# Autodesk Inventor assembly: Linear slides
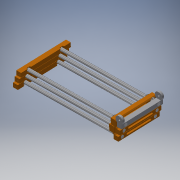
[picture p0: Inventor's stored thumbnail of the model, 180x180]
Saved by Autodesk Inventor 2019 (Build 230136000, 136)
## iProperties
Created: 2019-03-07
Part Number: Linear slides
Document SubType Name: Assembly
Designer: Delta
Mass: 697.362 g
Surface Area: 1389.66 cm^2
Volume: 258.282 cm^3
Density: 2.7 g/cm^3
Author: Delta
## Documents named in this file (6)
- C:\Robotics\2019-20_CAD\Linear Slides\Linear slides.iam
- C:\Robotics\2019-20_CAD\Linear Slides\Block_3-8.ipt
- C:\Robotics\2019-20_CAD\Linear Slides\rod_3-8_12 inch.ipt
- C:\Robotics\COTSParts\Bearings - McMaster\60595K120_FIXED ALIGNMENT  LINEAR BALL BRNG.ipt
- C:\Robotics\2019-20_CAD\Linear Slides\axil mount.ipt
- C:\Robotics\2019-20_CAD\Linear Slides\end piece.ipt
## Components (16 placed, 5 different names)
1. Block_3-8:1 — Mate:3, Mate:4, Mate:9, Mate:11, Mate:13, Mate:14, Mate:20
2. Block_3-8:2 — Mate:5, Mate:6, Mate:10, Mate:12, Mate:17, Mate:18, Mate:23, Mate:24
3. rod_3-8_12 inch:1 — Mate:4, Mate:11, Mate:27, Insert:5
4. rod_3-8_12 inch:2 — Mate:5, Mate:10, Insert:1
5. rod_3-8_12 inch:3 — Mate:3, Mate:9, Mate:28, Insert:4
6. rod_3-8_12 inch:4 — Mate:6, Mate:12, Mate:32, Flush:5
7. rod_3-8_12 inch:5 — Mate:25, Flush:2, Mate:30, Insert:3
8. 60595K120_FIXED ALIGNMENT  LINEAR BALL BRNG:2 — Mate:13, Mate:26, Flush:1
9. 60595K120_FIXED ALIGNMENT  LINEAR BALL BRNG:4 — Mate:14, Mate:20, Mate:25, Flush:1, Mate:33
10. 60595K120_FIXED ALIGNMENT  LINEAR BALL BRNG:5 — Mate:17, Mate:23, Mate:28
11. 60595K120_FIXED ALIGNMENT  LINEAR BALL BRNG:6 — Mate:18, Mate:24, Mate:27, Mate:34
12. axil mount:1 — Mate:29, Flush:2, Flush:3, Mate:30
13. end piece:1 — Mate:32, Flush:5, Insert:1
14. end piece:2 — Insert:4, Insert:5, Mate:34
15. end piece:3 — Insert:2, Insert:3, Mate:33
16. rod_3-8_12 inch:6 — Mate:26, Mate:29, Flush:3, Insert:2
## Relationships (33: Mate 24, Insert 5, Flush 4)
- Mate:3: Block_3-8:1 ↔ rod_3-8_12 inch:3
- Mate:4: Block_3-8:1 ↔ rod_3-8_12 inch:1
- Mate:5: Block_3-8:2 ↔ rod_3-8_12 inch:2
- Mate:6: Block_3-8:2 ↔ rod_3-8_12 inch:4
- Mate:9: Block_3-8:1 ↔ rod_3-8_12 inch:3
- Mate:10: Block_3-8:2 ↔ rod_3-8_12 inch:2
- Mate:11: Block_3-8:1 ↔ rod_3-8_12 inch:1
- Mate:12: Block_3-8:2 ↔ rod_3-8_12 inch:4
- Mate:13: Block_3-8:1 ↔ 60595K120_FIXED ALIGNMENT  LINEAR BALL BRNG:2
- Mate:14: Block_3-8:1 ↔ 60595K120_FIXED ALIGNMENT  LINEAR BALL BRNG:4
- Mate:17: Block_3-8:2 ↔ 60595K120_FIXED ALIGNMENT  LINEAR BALL BRNG:5
- Mate:18: Block_3-8:2 ↔ 60595K120_FIXED ALIGNMENT  LINEAR BALL BRNG:6
- Mate:20: Block_3-8:1 ↔ 60595K120_FIXED ALIGNMENT  LINEAR BALL BRNG:4
- Mate:23: Block_3-8:2 ↔ 60595K120_FIXED ALIGNMENT  LINEAR BALL BRNG:5
- Mate:24: Block_3-8:2 ↔ 60595K120_FIXED ALIGNMENT  LINEAR BALL BRNG:6
- Mate:25: rod_3-8_12 inch:5 ↔ 60595K120_FIXED ALIGNMENT  LINEAR BALL BRNG:4
- Mate:26: 60595K120_FIXED ALIGNMENT  LINEAR BALL BRNG:2 ↔ rod_3-8_12 inch:6
- Mate:27: rod_3-8_12 inch:1 ↔ 60595K120_FIXED ALIGNMENT  LINEAR BALL BRNG:6
- Mate:28: rod_3-8_12 inch:3 ↔ 60595K120_FIXED ALIGNMENT  LINEAR BALL BRNG:5
- Flush:1: 60595K120_FIXED ALIGNMENT  LINEAR BALL BRNG:2 ↔ 60595K120_FIXED ALIGNMENT  LINEAR BALL BRNG:4
- Mate:29: axil mount:1 ↔ rod_3-8_12 inch:6
- Flush:2: rod_3-8_12 inch:5 ↔ axil mount:1
- Flush:3: axil mount:1 ↔ rod_3-8_12 inch:6
- Mate:30: rod_3-8_12 inch:5 ↔ axil mount:1
- Mate:32: rod_3-8_12 inch:4 ↔ end piece:1
- Flush:5: rod_3-8_12 inch:4 ↔ end piece:1
- Insert:1: rod_3-8_12 inch:2 ↔ end piece:1
- Insert:2: end piece:3 ↔ rod_3-8_12 inch:6
- Insert:3: rod_3-8_12 inch:5 ↔ end piece:3
- Insert:4: rod_3-8_12 inch:3 ↔ end piece:2
- Insert:5: rod_3-8_12 inch:1 ↔ end piece:2
- Mate:33: 60595K120_FIXED ALIGNMENT  LINEAR BALL BRNG:4 ↔ end piece:3
- Mate:34: 60595K120_FIXED ALIGNMENT  LINEAR BALL BRNG:6 ↔ end piece:2
